# Autodesk Inventor assembly: Frame 1682207302696
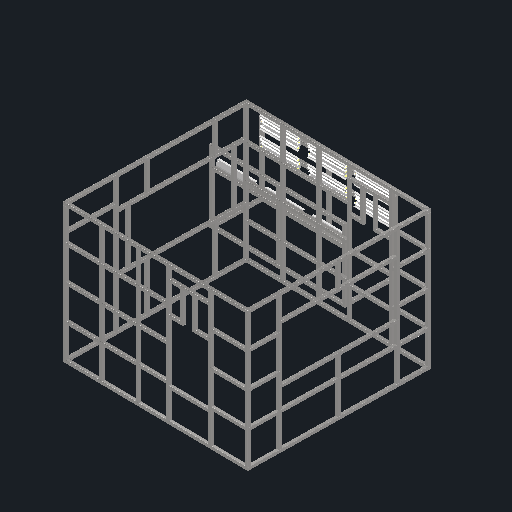
[picture p0: Inventor's stored thumbnail of the model, 512x512]
Saved by Autodesk Inventor 2024 (Build 280153000, 153)
## iProperties
Created: 2023-04-22
Part Number: Frame 1682207302696
Document SubType Name: Assembly
Designer: javie
_FrameDoc: Frame Assembly
_Version: 25.0.0
Author: javie
## Documents named in this file (85)
- C:\Users\javie\Downloads\Celda_Robotizada\Frame\Frame 1682207302696.iam
- C:\Users\javie\Downloads\Celda_Robotizada\Frame\Skeleton 1682207302718.ipt
- C:\Users\javie\Downloads\Celda_Robotizada\Frame\AISC 2 x 2 x 1_8 1682207398811.ipt
- C:\Users\javie\Downloads\Celda_Robotizada\Frame\AISC 2 x 2 x 1_8 1682207398853.ipt
- C:\Users\javie\Downloads\Celda_Robotizada\Frame\AISC 2 x 2 x 1_8 1682207398901.ipt
- C:\Users\javie\Downloads\Celda_Robotizada\Frame\AISC 2 x 2 x 1_8 1682207398943.ipt
- C:\Users\javie\Downloads\Celda_Robotizada\Frame\AISC 2 x 2 x 1_8 1682207398984.ipt
- C:\Users\javie\Downloads\Celda_Robotizada\Frame\AISC 2 x 2 x 1_8 1682207399024.ipt
- C:\Users\javie\Downloads\Celda_Robotizada\Frame\AISC 2 x 2 x 1_8 1682207399070.ipt
- C:\Users\javie\Downloads\Celda_Robotizada\Frame\AISC 2 x 2 x 1_8 1682207399113.ipt
- C:\Users\javie\Downloads\Celda_Robotizada\Frame\AISC 2 x 2 x 1_8 1682207399158.ipt
- C:\Users\javie\Downloads\Celda_Robotizada\Frame\AISC 2 x 2 x 1_8 1682207399200.ipt
- C:\Users\javie\Downloads\Celda_Robotizada\Frame\AISC 2 x 2 x 1_8 1682207399246.ipt
- C:\Users\javie\Downloads\Celda_Robotizada\Frame\AISC 2 x 2 x 1_8 1682207399287.ipt
- C:\Users\javie\Downloads\Celda_Robotizada\Frame\AISC 2 x 2 x 1_8 1682207399333.ipt
- C:\Users\javie\Downloads\Celda_Robotizada\Frame\AISC 2 x 2 x 1_8 1682207399378.ipt
- C:\Users\javie\Downloads\Celda_Robotizada\Frame\AISC 2 x 2 x 1_8 1682207399423.ipt
- C:\Users\javie\Downloads\Celda_Robotizada\Frame\AISC 2 x 2 x 1_8 1682207399464.ipt
- C:\Users\javie\Downloads\Celda_Robotizada\Frame\AISC 2 x 2 x 1_8 1682207399505.ipt
- C:\Users\javie\Downloads\Celda_Robotizada\Frame\AISC 2 x 2 x 1_8 1682207399546.ipt
- C:\Users\javie\Downloads\Celda_Robotizada\Frame\AISC 2 x 2 x 1_8 1682207399589.ipt
- C:\Users\javie\Downloads\Celda_Robotizada\Frame\AISC 2 x 2 x 1_8 1682207399630.ipt
- C:\Users\javie\Downloads\Celda_Robotizada\Frame\AISC 2 x 2 x 1_8 1682207399671.ipt
- C:\Users\javie\Downloads\Celda_Robotizada\Frame\AISC 2 x 2 x 1_8 1682207399711.ipt
- C:\Users\javie\Downloads\Celda_Robotizada\Frame\AISC 2 x 2 x 1_8 1682207399752.ipt
- C:\Users\javie\Downloads\Celda_Robotizada\Frame\AISC 2 x 2 x 1_8 1682207399795.ipt
- C:\Users\javie\Downloads\Celda_Robotizada\Frame\AISC 2 x 2 x 1_8 1682207399837.ipt
- C:\Users\javie\Downloads\Celda_Robotizada\Frame\AISC 2 x 2 x 1_8 1682207399879.ipt
- C:\Users\javie\Downloads\Celda_Robotizada\Frame\AISC 2 x 2 x 1_8 1682207399921.ipt
- C:\Users\javie\Downloads\Celda_Robotizada\Frame\AISC 2 x 2 x 1_8 1682207399966.ipt
- C:\Users\javie\Downloads\Celda_Robotizada\Frame\AISC 2 x 2 x 1_8 1682207400010.ipt
- C:\Users\javie\Downloads\Celda_Robotizada\Frame\AISC 2 x 2 x 1_8 1682207400053.ipt
- C:\Users\javie\Downloads\Celda_Robotizada\Frame\AISC 2 x 2 x 1_8 1682207400094.ipt
- C:\Users\javie\Downloads\Celda_Robotizada\Frame\AISC 2 x 2 x 1_8 1682207400138.ipt
- C:\Users\javie\Downloads\Celda_Robotizada\Frame\AISC 2 x 2 x 1_8 1682207400180.ipt
- C:\Users\javie\Downloads\Celda_Robotizada\Frame\AISC 2 x 2 x 1_8 1682207400222.ipt
- C:\Users\javie\Downloads\Celda_Robotizada\Frame\AISC 2 x 2 x 1_8 1682207400263.ipt
- C:\Users\javie\Downloads\Celda_Robotizada\Frame\AISC 2 x 2 x 1_8 1682207400307.ipt
- C:\Users\javie\Downloads\Celda_Robotizada\Frame\AISC 2 x 2 x 1_8 1682207400348.ipt
- C:\Users\javie\Downloads\Celda_Robotizada\Frame\AISC 2 x 2 x 1_8 1682207400391.ipt
- C:\Users\javie\Downloads\Celda_Robotizada\Frame\AISC 2 x 2 x 1_8 1682207400433.ipt
- C:\Users\javie\Downloads\Celda_Robotizada\Frame\AISC 2 x 2 x 1_8 1682207400476.ipt
- C:\Users\javie\Downloads\Celda_Robotizada\Frame\AISC 2 x 2 x 1_8 1682207400517.ipt
- C:\Users\javie\Downloads\Celda_Robotizada\Frame\AISC 2 x 2 x 1_8 1682207400559.ipt
- C:\Users\javie\Downloads\Celda_Robotizada\Frame\AISC 2 x 2 x 1_8 1682207400601.ipt
- C:\Users\javie\Downloads\Celda_Robotizada\Frame\AISC 2 x 2 x 1_8 1682207400648.ipt
- C:\Users\javie\Downloads\Celda_Robotizada\Frame\AISC 2 x 2 x 1_8 1682207400692.ipt
- C:\Users\javie\Downloads\Celda_Robotizada\Frame\AISC 2 x 2 x 1_8 1682207400745.ipt
- C:\Users\javie\Downloads\Celda_Robotizada\Frame\AISC 2 x 2 x 1_8 1682207400789.ipt
- C:\Users\javie\Downloads\Celda_Robotizada\Frame\AISC 2 x 2 x 1_8 1682207400831.ipt
- C:\Users\javie\Downloads\Celda_Robotizada\Frame\AISC 2 x 2 x 1_8 1682207400874.ipt
- C:\Users\javie\Downloads\Celda_Robotizada\Frame\AISC 2 x 2 x 1_8 1682207400916.ipt
- C:\Users\javie\Downloads\Celda_Robotizada\Frame\AISC 2 x 2 x 1_8 1682207400957.ipt
- C:\Users\javie\Downloads\Celda_Robotizada\Frame\AISC 2 x 2 x 1_8 1682207401000.ipt
- C:\Users\javie\Downloads\Celda_Robotizada\Frame\AISC 2 x 2 x 1_8 1682207401043.ipt
- C:\Users\javie\Downloads\Celda_Robotizada\Frame\AISC 2 x 2 x 1_8 1682207401087.ipt
- C:\Users\javie\Downloads\Celda_Robotizada\Frame\AISC 2 x 2 x 1_8 1682207401131.ipt
- C:\Users\javie\Downloads\Celda_Robotizada\Frame\AISC 2 x 2 x 1_8 1682207401172.ipt
- C:\Users\javie\Downloads\Celda_Robotizada\Frame\AISC 2 x 2 x 1_8 1682207401216.ipt
- C:\Users\javie\Downloads\Celda_Robotizada\Frame\AISC 2 x 2 x 1_8 1682207401258.ipt
- C:\Users\javie\Downloads\Celda_Robotizada\Frame\AISC 2 x 2 x 1_8 1682207401300.ipt
- C:\Users\javie\Downloads\Celda_Robotizada\Frame\AISC 2 x 2 x 1_8 1682207401342.ipt
- C:\Users\javie\Downloads\Celda_Robotizada\Frame\AISC 2 x 2 x 1_8 1682207401427.ipt
- C:\Users\javie\Downloads\Celda_Robotizada\Frame\AISC 2 x 2 x 1_8 1682207401469.ipt
- C:\Users\javie\Downloads\Celda_Robotizada\Frame\AISC 2 x 2 x 1_8 1682207401513.ipt
- C:\Users\javie\Downloads\Celda_Robotizada\Frame\AISC 2 x 2 x 1_8 1682207401557.ipt
- C:\Users\javie\Downloads\Celda_Robotizada\Frame\AISC 2 x 2 x 1_8 1682207401598.ipt
- C:\Users\javie\Downloads\Celda_Robotizada\Frame\AISC 2 x 2 x 1_8 1682207401639.ipt
- C:\Users\javie\Downloads\Celda_Robotizada\Frame\AISC 2 x 2 x 1_8 1682207401681.ipt
- C:\Users\javie\Downloads\Celda_Robotizada\Frame\AISC 2 x 2 x 1_8 1682207733021.ipt
- C:\Users\javie\Downloads\Celda_Robotizada\Frame\AISC 2 x 2 x 1_8 1682231625376.ipt
- C:\Users\javie\Downloads\Celda_Robotizada\Frame\AISC 2 x 2 x 1_8 1682231625424.ipt
- C:\Users\javie\Downloads\Celda_Robotizada\Frame\AISC 2 x 2 x 1_8 1682231625464.ipt
- C:\Users\javie\Downloads\Celda_Robotizada\Frame\AISC 2 x 2 x 1_8 1682231625506.ipt
- C:\Users\javie\Downloads\Celda_Robotizada\Frame\AISC 2 x 2 x 1_8 1682231625547.ipt
- C:\Users\javie\Downloads\Celda_Robotizada\Frame\AISC 2 x 2 x 1_8 1682231625589.ipt
- C:\Users\javie\Downloads\Celda_Robotizada\Frame\AISC 2 x 2 x 1_8 1682231625635.ipt
- C:\Users\javie\Downloads\Celda_Robotizada\Frame\AISC 2 x 2 x 1_8 1682231625676.ipt
- C:\Users\javie\Downloads\Celda_Robotizada\Frame\AISC 2 x 2 x 1_8 1682231625717.ipt
- C:\Users\javie\Downloads\Celda_Robotizada\Frame\AISC 2 x 2 x 1_8 1682231625759.ipt
- C:\Users\javie\Downloads\Celda_Robotizada\Frame\AISC 2 x 2 x 1_8 1682231672707.ipt
- C:\Users\javie\Downloads\Celda_Robotizada\Frame\AISC 2 x 2 x 1_8 1682231672749.ipt
- C:\Users\javie\Downloads\Celda_Robotizada\Frame\AISC 2 x 2 x 1_8 1682231672791.ipt
- C:\Users\javie\Downloads\Celda_Robotizada\Frame\AISC 2 x 2 x 1_8 1682231672833.ipt
- C:\Users\javie\Downloads\Celda de Manufactura\LamparaSe.iam
## Components (92 placed, 28 different names)
1. Reference Skeleton
2. AISC 2 x 2 x 1/8 - 84,614:1
3. AISC 2 x 2 x 1/8 - 120,11:1
4. AISC 2 x 2 x 1/8 - 120,11:2
5. AISC 2 x 2 x 1/8 - 84,614:2
6. AISC 2 x 2 x 1/8 - 66,929:1
7. AISC 2 x 2 x 1/8 - 66,929:2
8. AISC 2 x 2 x 1/8 - 66,929:3
9. AISC 2 x 2 x 1/8 - 84,614:3
10. AISC 2 x 2 x 1/8 - 84,614:4
11. AISC 2 x 2 x 1/8 - 27,559:1
12. AISC 2 x 2 x 1/8 - 84,614:5
13. AISC 2 x 2 x 1/8 - 84,614:6
14. AISC 2 x 2 x 1/8 - 23,622:1
15. AISC 2 x 2 x 1/8 - 23,622:2
16. AISC 2 x 2 x 1/8 - 23,622:3
17. AISC 2 x 2 x 1/8 - 11,63:1
18. AISC 2 x 2 x 1/8 - 20,685:1
19. AISC 2 x 2 x 1/8 - 20,685:2
20. AISC 2 x 2 x 1/8 - 10,055:1
21. AISC 2 x 2 x 1/8 - 27,559:2
22. AISC 2 x 2 x 1/8 - 115,78:1
23. AISC 2 x 2 x 1/8 - 113,78:2
24. AISC 2 x 2 x 1/8 - 74,409:1
25. AISC 2 x 2 x 1/8 - 74,409:2
26. AISC 2 x 2 x 1/8 - 115,78:3
27. AISC 2 x 2 x 1/8 - 19,685:3
28. AISC 2 x 2 x 1/8 - 19,685:4
29. AISC 2 x 2 x 1/8 - 84,614:7
30. AISC 2 x 2 x 1/8 - 14,748:1
31. AISC 2 x 2 x 1/8 - 34,433:1
32. AISC 2 x 2 x 1/8 - 19,685:5
33. AISC 2 x 2 x 1/8 - 19,685:6
34. AISC 2 x 2 x 1/8 - 84,614:8
35. AISC 2 x 2 x 1/8 - 120,11:3
36. AISC 2 x 2 x 1/8 - 23,622:4
37. AISC 2 x 2 x 1/8 - 23,622:5
38. AISC 2 x 2 x 1/8 - 23,622:6
39. AISC 2 x 2 x 1/8 - 120,11:4
40. AISC 2 x 2 x 1/8 - 84,614:9
41. AISC 2 x 2 x 1/8 - 27,559:3
42. AISC 2 x 2 x 1/8 - 11,63:2
43. AISC 2 x 2 x 1/8 - 27,559:4
44. AISC 2 x 2 x 1/8 - 20,685:7
45. AISC 2 x 2 x 1/8 - 20,685:8
46. AISC 2 x 2 x 1/8 - 10,055:2
47. AISC 2 x 2 x 1/8 - 84,614:10
48. AISC 2 x 2 x 1/8 - 66,929:4
49. AISC 2 x 2 x 1/8 - 66,929:5
50. AISC 2 x 2 x 1/8 - 66,929:6
51. AISC 2 x 2 x 1/8 - 84,614:11
52. AISC 2 x 2 x 1/8 - 84,614:12
53. AISC 2 x 2 x 1/8 - 85,614:13
54. AISC 2 x 2 x 1/8 - 115,78:4
55. AISC 2 x 2 x 1/8 - 84,614:14
56. AISC 2 x 2 x 1/8 - 84,614:15
57. AISC 2 x 2 x 1/8 - 115,78:5
58. AISC 2 x 2 x 1/8 - 29,496:1
59. AISC 2 x 2 x 1/8 - 69,866:1
60. AISC 2 x 2 x 1/8 - 14,748:2
61. AISC 2 x 2 x 1/8 - 80,283:1
62. AISC 2 x 2 x 1/8 - 80,283:2
63. AISC 2 x 2 x 1/8 - 33,433:2
64. AISC 2 x 2 x 1/8 - 17,685:9
65. AISC 2 x 2 x 1/8 - 29,496:1
66. AISC 2 x 2 x 1/8 - 17,685:10
67. AISC 2 x 2 x 1/8 - 29,496:2
68. AISC 2 x 2 x 1/8 - 33,433:3
69. AISC 2 x 2 x 1/8 - 84,614:16
70. AISC 2 x 2 x 1/8 - 46,202:1
71. AISC 2 x 2 x 1/8 - 88,22:1
72. AISC 2 x 2 x 1/8 - 86,22:2 — Insertar:1, Insertar:2, Insertar:3
73. AISC 2 x 2 x 1/8 - 45,276:2
74. AISC 2 x 2 x 1/8 - 46,202:3
75. AISC 2 x 2 x 1/8 - 86,22:3 — Insertar:4, Insertar:5, Insertar:6
76. AISC 2 x 2 x 1/8 - 88,22:4 — Insertar:7, Insertar:8, Insertar:9
77. AISC 2 x 2 x 1/8 - 46,202:4
78. AISC 2 x 2 x 1/8 - 45,276:5
79. AISC 2 x 2 x 1/8 - 46,202:6
80. AISC 2 x 2 x 1/8 - 88,074:5
81. AISC 2 x 2 x 1/8 - 33,35:3
82. AISC 2 x 2 x 1/8 - 88,074:6
83. AISC 2 x 2 x 1/8 - 33,35:4
84. LamparaSe:1 [sub-assembly] — Insertar:3
85. LamparaSe:2 [sub-assembly] — Insertar:2
86. LamparaSe:3 [sub-assembly] — Insertar:1
87. LamparaSe:4 [sub-assembly] — Insertar:4
88. LamparaSe:5 [sub-assembly] — Insertar:8
89. LamparaSe:6 [sub-assembly] — Insertar:9
90. LamparaSe:7 [sub-assembly] — Insertar:7
91. LamparaSe:8 [sub-assembly] — Insertar:5
92. LamparaSe:9 [sub-assembly] — Insertar:6
## Relationships (9: Insert 9)
- Insertar:1: AISC 2 x 2 x 1/8 - 86,22:2 ↔ LamparaSe:3
- Insertar:2: AISC 2 x 2 x 1/8 - 86,22:2 ↔ LamparaSe:2
- Insertar:3: AISC 2 x 2 x 1/8 - 86,22:2 ↔ LamparaSe:1
- Insertar:4: AISC 2 x 2 x 1/8 - 86,22:3 ↔ LamparaSe:4
- Insertar:5: AISC 2 x 2 x 1/8 - 86,22:3 ↔ LamparaSe:8
- Insertar:6: AISC 2 x 2 x 1/8 - 86,22:3 ↔ LamparaSe:9
- Insertar:7: AISC 2 x 2 x 1/8 - 88,22:4 ↔ LamparaSe:7
- Insertar:8: AISC 2 x 2 x 1/8 - 88,22:4 ↔ LamparaSe:5
- Insertar:9: AISC 2 x 2 x 1/8 - 88,22:4 ↔ LamparaSe:6
